# Autodesk Inventor assembly: Assembly_components
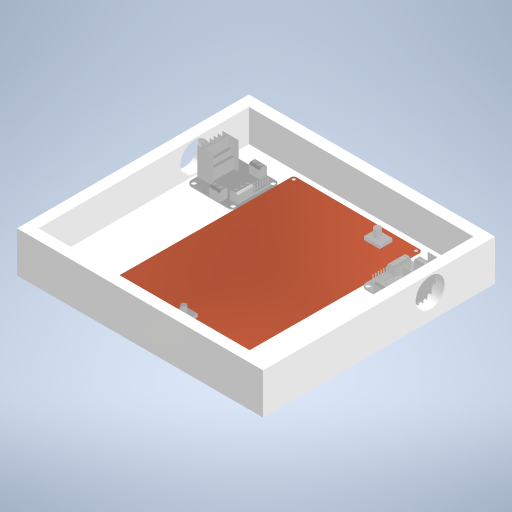
[picture p0: Inventor's stored thumbnail of the model, 512x512]
Saved by Autodesk Inventor 2023 (Build 270158000, 158)
## iProperties
Created: 2023-03-21
Part Number: Assembly_components
Document SubType Name: Assembly
Designer: 55119
Author: 55119
## Documents named in this file (4)
- C:\Users\55119\Documents\GitHub\tectonics\src\3d_models\Case\Assembly_components.iam
- C:\Users\55119\Documents\GitHub\tectonics\src\3d_models\Case\PCB.ipt
- C:\Users\55119\Documents\GitHub\tectonics\src\3d_models\Case\Ponte_H.ipt
- C:\Users\55119\Documents\GitHub\tectonics\src\3d_models\Case\Case_3d_model.ipt
## Components (4 placed, 3 different names)
1. PCB:1 — Mate:4, Mate:5, Mate:6, Mate:7, Mate:8
2. Ponte_H:1 — Mate:5, Mate:10
3. Ponte_H:2 — Mate:4, Mate:7, Mate:8, Mate:9
4. Case_3d_model:1 — Mate:6, Mate:9, Mate:10
## Relationships (7: Mate 7)
- Mate:4: PCB:1 ↔ Ponte_H:2
- Mate:5: PCB:1 ↔ Ponte_H:1
- Mate:6: PCB:1 ↔ Case_3d_model:1
- Mate:7: PCB:1 ↔ Ponte_H:2
- Mate:8: PCB:1 ↔ Ponte_H:2
- Mate:9: Ponte_H:2 ↔ Case_3d_model:1
- Mate:10: Ponte_H:1 ↔ Case_3d_model:1
